# Autodesk Inventor assembly: Ensamble EVA
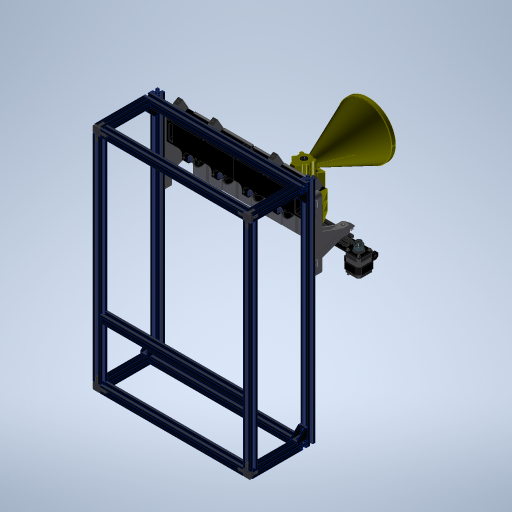
[picture p0: Inventor's stored thumbnail of the model, 512x512]
Saved by Autodesk Inventor 2023 (Build 270158000, 158)
## iProperties
Created: 2021-02-21
Part Number: Ensamble EVA
Document SubType Name: Assembly
Designer: juanp
Author: juanp
## Documents named in this file (11)
- C:\Users\juanp\OneDrive - Universidad de los andes\Uniandes\Robocol\EVA\V3 (Actual)\Ensamble EVA V3.iam
- C:\Users\juanp\OneDrive - Universidad de los andes\Uniandes\Robocol\EVA\Recursos\Actuador Lineal\Actuador Lineal (sin carro).iam
- C:\Users\juanp\OneDrive - Universidad de los andes\Uniandes\Robocol\EVA\Recursos\Chasis\Diseño 1.3 (2020)\Ensamble_chasis.iam
- C:\Users\juanp\OneDrive - Universidad de los andes\Uniandes\Robocol\EVA\Recursos\Actuador Lineal\Carro deslizante\Carro Deslizante.ipt
- C:\Users\juanp\OneDrive - Universidad de los andes\Uniandes\Robocol\EVA\V3 (Actual)\Dispensador\Dispensador V3.iam
- C:\Users\juanp\OneDrive - Universidad de los andes\Uniandes\Robocol\EVA\V3 (Actual)\Cajas\cajas_V3.iam
- C:\Users\juanp\OneDrive - Universidad de los andes\Uniandes\Robocol\EVA\V3 (Actual)\Acople a chasis\Soporte Cajas.ipt
- C:\Users\juanp\OneDrive - Universidad de los andes\Uniandes\Robocol\EVA\Recursos\Fin de carrera\Fin de carrera.ipt
- C:\Users\juanp\OneDrive - Universidad de los andes\Uniandes\Robocol\EVA\V3 (Actual)\Acople a chasis\Soporte ajustado a deflexion - fin de carrera.ipt
- C:\Users\juanp\OneDrive - Universidad de los andes\Uniandes\Robocol\EVA\V3 (Actual)\Acople a chasis\Soporte ajustado a deflexion.ipt
- C:\Users\juanp\OneDrive - Universidad de los andes\Uniandes\Robocol\EVA\V3 (Actual)\Acople a chasis\Montura motor para cadena.ipt
## Components (11 placed, 10 different names)
1. Actuador Lineal (sin carro):1 [sub-assembly] — Angle:1, Angle:2, Mate:1, Angle:3, Angle:4, Flush:2, Mate:3, Angle:5, Flush:4, Flush:13, Flush:14, Mate:89, Mate:90, Angle:6, Mate:91
2. Ensamble_chasis:1 [sub-assembly] — Angle:1, Angle:2, Mate:1, Mate:88, Flush:10, Flush:11, Flush:16
3. Carro Deslizante:1 — Angle:3, Angle:4, Flush:2, Mate:3, Mate:42, Mate:43, Mate:44
4. Dispensador V3:1 [sub-assembly] — Mate:42, Mate:43, Mate:44, Mate:69
5. cajas_V3:1 [sub-assembly] — Angle:5, Mate:88, Flush:4, Mate:53, Flush:7, Mate:54, Flush:8, Mate:69, Mate:70, Mate:75, Flush:16
6. Soporte Cajas:1 — Mate:53, Flush:7, Mate:70, Mate:92
7. Soporte Cajas:2 — Mate:54, Flush:8, Mate:75
8. Fin de carrera:1 — Mate:66, Mate:67, Mate:68
9. Soporte ajustado a deflexion - fin de carrera:1 — Flush:10, Mate:66, Mate:67, Mate:68, Flush:13, Flush:15, Mate:89, Mate:92
10. Soporte ajustado a deflexion:1 — Flush:11, Flush:14, Flush:15
11. Montura motor para cadena:1 — Mate:90, Angle:6, Mate:91
## Relationships (34: Mate 18, Flush 10, Angle 6)
- Angle:1 (180 deg): Actuador Lineal (sin carro):1 ↔ Ensamble_chasis:1
- Angle:2 (0 deg): Actuador Lineal (sin carro):1 ↔ Ensamble_chasis:1
- Mate:1: Actuador Lineal (sin carro):1 ↔ Ensamble_chasis:1
- Angle:3 (0 deg): Actuador Lineal (sin carro):1 ↔ Carro Deslizante:1
- Angle:4 (180 deg): Actuador Lineal (sin carro):1 ↔ Carro Deslizante:1
- Flush:2: Actuador Lineal (sin carro):1 ↔ Carro Deslizante:1
- Mate:3: Actuador Lineal (sin carro):1 ↔ Carro Deslizante:1
- Mate:42: Carro Deslizante:1 ↔ Dispensador V3:1
- Mate:43: Carro Deslizante:1 ↔ Dispensador V3:1
- Mate:44: Carro Deslizante:1 ↔ Dispensador V3:1
- Angle:5 (180 deg): Actuador Lineal (sin carro):1 ↔ cajas_V3:1
- Mate:88: Ensamble_chasis:1 ↔ cajas_V3:1
- Flush:4: Actuador Lineal (sin carro):1 ↔ cajas_V3:1
- Mate:53: cajas_V3:1 ↔ Soporte Cajas:1
- Flush:7: cajas_V3:1 ↔ Soporte Cajas:1
- Mate:54: cajas_V3:1 ↔ Soporte Cajas:2
- Flush:8: cajas_V3:1 ↔ Soporte Cajas:2
- Flush:10: Ensamble_chasis:1 ↔ Soporte ajustado a deflexion - fin de carrera:1
- Mate:66: Fin de carrera:1 ↔ Soporte ajustado a deflexion - fin de carrera:1
- Mate:67: Fin de carrera:1 ↔ Soporte ajustado a deflexion - fin de carrera:1
- Mate:68: Fin de carrera:1 ↔ Soporte ajustado a deflexion - fin de carrera:1
- Flush:11: Ensamble_chasis:1 ↔ Soporte ajustado a deflexion:1
- Flush:13 (-20 mm): Actuador Lineal (sin carro):1 ↔ Soporte ajustado a deflexion - fin de carrera:1
- Flush:14: Actuador Lineal (sin carro):1 ↔ Soporte ajustado a deflexion:1
- Flush:15: Soporte ajustado a deflexion - fin de carrera:1 ↔ Soporte ajustado a deflexion:1
- Mate:69 (3.5 mm): Dispensador V3:1 ↔ cajas_V3:1
- Mate:70: cajas_V3:1 ↔ Soporte Cajas:1
- Mate:75: cajas_V3:1 ↔ Soporte Cajas:2
- Mate:89: Actuador Lineal (sin carro):1 ↔ Soporte ajustado a deflexion - fin de carrera:1
- Flush:16 (64 mm): Ensamble_chasis:1 ↔ cajas_V3:1
- Mate:90: Actuador Lineal (sin carro):1 ↔ Montura motor para cadena:1
- Angle:6 (0 deg): Actuador Lineal (sin carro):1 ↔ Montura motor para cadena:1
- Mate:91: Actuador Lineal (sin carro):1 ↔ Montura motor para cadena:1
- Mate:92: Soporte Cajas:1 ↔ Soporte ajustado a deflexion - fin de carrera:1
